# Autodesk Inventor assembly: wheel sub assemblly trackshen wheel
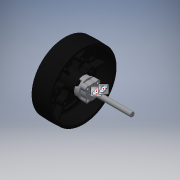
[picture p0: Inventor's stored thumbnail of the model, 180x180]
Saved by Autodesk Inventor 2017 (Build 210142000, 142)
## iProperties
Created: 2017-08-02
Part Number: wheel sub assemblly trackshen wheel
Document SubType Name: Assembly
Designer: User
Author: User
## Documents named in this file (6)
- C:\Robotics\CAD\2016-17_CAD\DriveTrain\wheel sub assemblly trackshen wheel.iam
- C:\Robotics\CAD\COTSParts\Wheels\4in Wheel Intergreated Hub 8mm Rev2.ipt
- C:\Robotics\CAD\COTSParts\Actobotics\634 parts\634080.ipt
- C:\Robotics\CAD\COTSParts\Actobotics\545 parts\545556.ipt
- C:\Robotics\CAD\COTSParts\Actobotics\545 parts\545456.ipt
- C:\Robotics\CAD\COTSParts\Actobotics\615 parts\615106.ipt
## Components (6 placed, 5 different names)
1. 4in Wheel Intergreated Hub 8mm Rev2:1 — Mate:1, Mate:6, Mate:10
2. 634080:1 — Mate:1, Mate:3, Mate:5, Mate:8
3. 545556:1 — Mate:2, Mate:8, Mate:9
4. 545556:2 — Mate:5, Mate:7
5. 545456:2 — Mate:3, Mate:6, Mate:7
6. 615106:1 — Mate:2, Mate:9, Mate:10
## Relationships (9: Mate 9)
- Mate:1: 4in Wheel Intergreated Hub 8mm Rev2:1 ↔ 634080:1
- Mate:2: 545556:1 ↔ 615106:1
- Mate:3: 634080:1 ↔ 545456:2
- Mate:5: 634080:1 ↔ 545556:2
- Mate:6: 4in Wheel Intergreated Hub 8mm Rev2:1 ↔ 545456:2
- Mate:7: 545556:2 ↔ 545456:2
- Mate:8: 634080:1 ↔ 545556:1
- Mate:9: 545556:1 ↔ 615106:1
- Mate:10 (6.35 mm): 4in Wheel Intergreated Hub 8mm Rev2:1 ↔ 615106:1
